# Autodesk Inventor assembly: omni wheels-26 tooth sproket
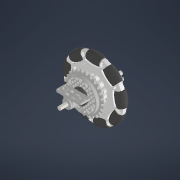
[picture p0: Inventor's stored thumbnail of the model, 180x180]
Saved by Autodesk Inventor 2022 (Build 260153000, 153)
## iProperties
Created: 2021-12-01
Part Number: omni wheels-26 tooth sproket
Document SubType Name: Assembly
Designer: izack
Author: izack
## Documents named in this file (7)
- F:\CAD Modeling\GithubCAD\ComputerAidedDesign\2021-22\FTC\#12456 Big Red\Drivetrain\Omni Wheel Drive\omni wheels-26 tooth sproket.iam
- F:\CAD Modeling\GithubCAD\ComputerAidedDesign\2021-22\FTC\Parts\REV Parts\90mm Omni Wheel - 2 Pack.ipt
- F:\CAD Modeling\GithubCAD\ComputerAidedDesign\2021-22\FTC\Parts\REV Parts\26 Tooth #25 Sprocket - 4 Pack.ipt
- F:\CAD Modeling\GithubCAD\ComputerAidedDesign\2021-22\FTC\Parts\REV Parts\High Strength Hex Hub - 2 Pack.ipt
- F:\CAD Modeling\GithubCAD\ComputerAidedDesign\2021-22\FTC\Parts\REV Parts\15mm Bearing Pillow Block - 8 Pack.ipt
- F:\CAD Modeling\GithubCAD\ComputerAidedDesign\2021-22\FTC\Parts\REV Parts\5mm x 90mm Hex Shaft - 4 Pack.ipt
- F:\CAD Modeling\GithubCAD\ComputerAidedDesign\2021-22\FTC\Parts\REV Parts\Through Bore Bearing - Short - 12 Pack.ipt
## Components (9 placed, 6 different names)
1. 90mm Omni Wheel - 2 Pack:1 — Mate:1, Mate:6, Mate:7, Mate:8, Mate:9, Mate:10, Mate:28
2. 26 Tooth #25 Sprocket - 4 Pack:1 — Mate:8, Mate:9, Mate:10, Mate:11, Mate:12
3. High Strength Hex Hub - 2 Pack:1 — Mate:11, Mate:12, Mate:13, Mate:14, Mate:28
4. High Strength Hex Hub - 2 Pack:7 — Mate:1, Mate:6, Mate:7, Mate:15, Mate:16, Mate:17, Mate:18
5. 15mm Bearing Pillow Block - 8 Pack:1 — Mate:13, Mate:14, Symmetry:1, Mate:23
6. 15mm Bearing Pillow Block - 8 Pack:2 — Mate:15, Mate:16, Symmetry:1, Mate:20
7. 5mm x 90mm Hex Shaft - 4 Pack:1 — Mate:17, Mate:18, Mate:19, Mate:21, Mate:22, Mate:24, Mate:25
8. Through Bore Bearing - Short - 12 Pack:1 — Mate:20, Mate:21, Mate:22
9. Through Bore Bearing - Short - 12 Pack:2 — Mate:23, Mate:24, Mate:25
## Relationships (23: Mate 22, Symmetry 1)
- Mate:1: 90mm Omni Wheel - 2 Pack:1 ↔ High Strength Hex Hub - 2 Pack:7
- Mate:6: 90mm Omni Wheel - 2 Pack:1 ↔ High Strength Hex Hub - 2 Pack:7
- Mate:7: 90mm Omni Wheel - 2 Pack:1 ↔ High Strength Hex Hub - 2 Pack:7
- Mate:8: 90mm Omni Wheel - 2 Pack:1 ↔ 26 Tooth #25 Sprocket - 4 Pack:1
- Mate:9: 90mm Omni Wheel - 2 Pack:1 ↔ 26 Tooth #25 Sprocket - 4 Pack:1
- Mate:10: 90mm Omni Wheel - 2 Pack:1 ↔ 26 Tooth #25 Sprocket - 4 Pack:1
- Mate:11: 26 Tooth #25 Sprocket - 4 Pack:1 ↔ High Strength Hex Hub - 2 Pack:1
- Mate:12: 26 Tooth #25 Sprocket - 4 Pack:1 ↔ High Strength Hex Hub - 2 Pack:1
- Mate:13: High Strength Hex Hub - 2 Pack:1 ↔ 15mm Bearing Pillow Block - 8 Pack:1
- Mate:14: High Strength Hex Hub - 2 Pack:1 ↔ 15mm Bearing Pillow Block - 8 Pack:1
- Mate:15: High Strength Hex Hub - 2 Pack:7 ↔ 15mm Bearing Pillow Block - 8 Pack:2
- Mate:16: High Strength Hex Hub - 2 Pack:7 ↔ 15mm Bearing Pillow Block - 8 Pack:2
- Mate:17: High Strength Hex Hub - 2 Pack:7 ↔ 5mm x 90mm Hex Shaft - 4 Pack:1
- Mate:18: High Strength Hex Hub - 2 Pack:7 ↔ 5mm x 90mm Hex Shaft - 4 Pack:1
- Symmetry:1: 15mm Bearing Pillow Block - 8 Pack:1 ↔ 15mm Bearing Pillow Block - 8 Pack:2
- Mate:19 (-45 mm): 5mm x 90mm Hex Shaft - 4 Pack:1
- Mate:20: 15mm Bearing Pillow Block - 8 Pack:2 ↔ Through Bore Bearing - Short - 12 Pack:1
- Mate:21: 5mm x 90mm Hex Shaft - 4 Pack:1 ↔ Through Bore Bearing - Short - 12 Pack:1
- Mate:22: 5mm x 90mm Hex Shaft - 4 Pack:1 ↔ Through Bore Bearing - Short - 12 Pack:1
- Mate:23: 15mm Bearing Pillow Block - 8 Pack:1 ↔ Through Bore Bearing - Short - 12 Pack:2
- Mate:24: 5mm x 90mm Hex Shaft - 4 Pack:1 ↔ Through Bore Bearing - Short - 12 Pack:2
- Mate:25: 5mm x 90mm Hex Shaft - 4 Pack:1 ↔ Through Bore Bearing - Short - 12 Pack:2
- Mate:28: 90mm Omni Wheel - 2 Pack:1 ↔ High Strength Hex Hub - 2 Pack:1
